# Autodesk Inventor assembly: HAND_asm2
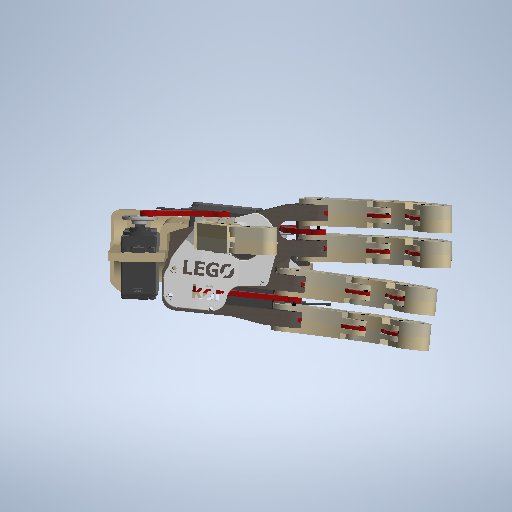
[picture p0: Inventor's stored thumbnail of the model, 512x512]
Saved by Autodesk Inventor 2025.2 (Build 292293000, 293)
## iProperties
Part Number: HAND_asm2
Document SubType Name: Assembly
Designer: esandor
Author: esandor
## Documents named in this file (23)
- C:\Users\esandor\Documents\Inventor\INDACT_EE\again\HAND_THIS_IS_IT.iam
- C:\Users\esandor\Documents\Inventor\INDACT_EE\again\PALM\PALM_base.ipt
- C:\Users\esandor\Documents\Inventor\INDACT_EE\again\HAND\HAND_double_finger_dowel_pin.ipt
- C:\Users\esandor\Documents\Inventor\INDACT_EE\again\FINGER\FIN_phalanx_proximal_top.ipt
- C:\Users\esandor\Documents\Inventor\INDACT_EE\again\FINGER\FIN_dowel_pin_long.ipt
- C:\Users\esandor\Documents\Inventor\INDACT_EE\again\FINGER\FIN_phalanx_proximal_base.ipt
- C:\Users\esandor\Documents\Inventor\INDACT_EE\again\FINGER\FIN_phalanx_media_top.ipt
- C:\Users\esandor\Documents\Inventor\INDACT_EE\again\FINGER\FIN_phalanx_media_base.ipt
- C:\Users\esandor\Documents\Inventor\INDACT_EE\again\FINGER\FIN_dowel_pin_short.ipt
- C:\Users\esandor\Documents\Inventor\INDACT_EE\again\FINGER\FIN_phalanx_distal_top.ipt
- C:\Users\esandor\Documents\Inventor\INDACT_EE\again\FINGER\FIN_phalanx_distal_base.ipt
- C:\Users\esandor\Documents\Inventor\INDACT_EE\again\FINGER\FIN_mech_proximal.ipt
- C:\Users\esandor\Documents\Inventor\INDACT_EE\again\FINGER\FIN_mech_distal.ipt
- C:\Users\esandor\Documents\Inventor\INDACT_EE\again\PALM\PALM_logo.ipt
- C:\Users\esandor\Documents\Inventor\INDACT_EE\again\PALM\PALM_lower_motor_holder.ipt
- C:\Users\esandor\Documents\Inventor\INDACT_EE\again\PALM\PALM_upper_motor_holder.ipt
- C:\Users\esandor\Documents\Inventor\INDACT_EE\again\HAND\HAND_motor_base.ipt
- C:\Users\esandor\Documents\Inventor\INDACT_EE\again\HAND\HAND_motor_top.ipt
- C:\Users\esandor\Documents\Inventor\INDACT_EE\again\HAND\HAND_gyuru.ipt
- C:\Users\esandor\Documents\Inventor\INDACT_EE\again\HAND\HAND_nut.ipt
- C:\Users\esandor\Documents\Inventor\INDACT_EE\again\HAND\HAND_mech_little_finger.ipt
- C:\Users\esandor\Documents\Inventor\INDACT_EE\again\HAND\HAND_mech_thumb_finger.ipt
- C:\Users\esandor\Documents\Inventor\INDACT_EE\again\HAND\HAND_mech_index_finger.ipt
## Components (81 placed, 22 different names)
1. PALM_base:1 — Mate:2, Tangent:2, Insert:2, Insert:9, Insert:11, Mate:24, Tangent:44, Mate:25, Insert:30, Insert:31, Mate:28, Insert:32, Insert:33, Tangent:63, Mate:36, Insert:42, Insert:43, Mate:37, Insert:44, Insert:45
2. FIN_dowel_pin_short:1 — Insert:2, Tangent:5
3. FIN_phalanx_proximal_top:1 — Mate:1, Insert:1, Tangent:1, Mate:2, Tangent:2, Insert:4, Mate:4, Insert:5, Mate:5
4. FIN_phalanx_proximal_base:1 — Mate:1, Insert:1, Tangent:1, Tangent:21
5. FIN_dowel_pin_short:2 — Insert:4, Tangent:9
6. FIN_phalanx_media_top:1 — Mate:3, Tangent:3, Tangent:4, Mate:4, Insert:5, Insert:6, Insert:7, Mate:7
7. FIN_phalanx_media_base:1 — Mate:3, Tangent:3, Tangent:4, Angle:1
8. FIN_dowel_pin_long:2 — Insert:6, Tangent:6
9. FIN_mech_proximal:1 — Tangent:5, Mate:5, Tangent:6
10. FIN_phalanx_distal_top:1 — Mate:6, Tangent:7, Tangent:8, Insert:7, Insert:8
11. FIN_phalanx_distal_base:1 — Mate:6, Tangent:7, Tangent:8, Angle:2
12. FIN_dowel_pin_long:3 — Insert:8, Tangent:10
13. FIN_mech_distal:1 — Mate:7, Tangent:9, Tangent:10
14. FIN_phalanx_proximal_top:2 — Tangent:11, Tangent:12, Mate:8, Insert:9, Insert:12, Insert:13, Mate:10, Insert:17
15. FIN_phalanx_proximal_base:2 — Tangent:11, Tangent:12, Mate:8, Mate:49
16. FIN_dowel_pin_short:3 — Insert:11, Tangent:15
17. FIN_dowel_pin_short:4 — Insert:12, Tangent:19
18. FIN_phalanx_media_top:2 — Insert:13, Insert:14, Insert:15, Mate:12
19. FIN_phalanx_media_base:2 — Angle:1
20. FIN_dowel_pin_long:5 — Insert:14, Tangent:16
21. FIN_mech_proximal:2 — Mate:10, Tangent:15, Tangent:16
22. FIN_phalanx_distal_top:2 — Insert:15, Insert:16
23. FIN_phalanx_distal_base:2 — Angle:2
24. FIN_dowel_pin_long:6 — Insert:16, Tangent:20
25. FIN_mech_distal:3 — Tangent:19, Mate:12, Tangent:20
26. HAND_double_finger_dowel_pin:3 — Insert:17, Tangent:21, Tangent:65
27. FIN_phalanx_proximal_top:3 — Mate:25, Mate:26, Mate:52
28. FIN_phalanx_proximal_base:3 — Tangent:63
29. FIN_dowel_pin_short:6
30. FIN_phalanx_media_top:3
31. FIN_phalanx_media_base:3
32. FIN_dowel_pin_long:7 — Tangent:48
33. FIN_phalanx_distal_top:3
34. FIN_phalanx_distal_base:3
35. FIN_dowel_pin_long:8
36. FIN_mech_distal:4
37. FIN_phalanx_proximal_top:4 — Mate:24, Tangent:44, Mate:27
38. FIN_phalanx_proximal_base:4
39. FIN_dowel_pin_short:8
40. FIN_phalanx_media_top:4
41. FIN_phalanx_media_base:4
42. FIN_dowel_pin_long:9 — Tangent:50
43. FIN_phalanx_distal_top:4
44. FIN_phalanx_distal_base:4
45. FIN_dowel_pin_long:10
46. FIN_mech_distal:5
47. HAND_double_finger_dowel_pin:4 — Tangent:67
48. FIN_dowel_pin_short:9 — Insert:30, Tangent:47
49. FIN_mech_proximal:3 — Mate:26, Tangent:47, Tangent:48
50. FIN_dowel_pin_short:10 — Insert:31, Tangent:49
51. FIN_mech_proximal:4 — Mate:27, Tangent:49, Tangent:50
52. PALM_logo:1 — Mate:28, Insert:32, Insert:33, Mate:35, Insert:40, Insert:41
53. FIN_phalanx_proximal_top:5 — Insert:54
54. FIN_phalanx_proximal_base:5 — Mate:35, Insert:40
55. FIN_dowel_pin_short:12
56. FIN_phalanx_media_top:5
57. FIN_phalanx_media_base:5
58. FIN_dowel_pin_long:11
59. FIN_mech_proximal:5 — Tangent:62
60. FIN_phalanx_distal_top:5
61. FIN_phalanx_distal_base:5
62. FIN_dowel_pin_long:12
63. FIN_mech_distal:6
64. FIN_dowel_pin_short:13 — Insert:41, Tangent:62
65. PALM_lower_motor_holder:1 — Mate:36, Insert:42, Insert:43, Mate:40, Insert:55, Insert:56
66. PALM_upper_motor_holder:1 — Mate:37, Insert:44, Insert:45, Mate:38, Insert:46, Insert:47, Mate:39, Insert:48, Insert:49
67. HAND_motor_base:1 — Mate:38, Insert:46, Insert:47, Rotational:2
68. HAND_motor_base:2 — Mate:39, Insert:48, Insert:49, Rotational:1
69. HAND_motor_base:3 — Mate:40, Insert:55, Insert:56, Rotational:3
70. HAND_motor_top:1 — Rotational:1, Tangent:70
71. HAND_gyuru:1 — Tangent:64, Flush:1, Tangent:65
72. HAND_nut:1 — Mate:50, Mate:51, Tangent:68
73. HAND_mech_little_finger:1 — Mate:50, Mate:51, Tangent:66, Flush:2, Mate:52
74. HAND_mech_thumb_finger:1 — Mate:44, Mate:45, Mate:46, Tangent:71
75. HAND_nut:2 — Mate:44, Tangent:70, Tangent:71
76. HAND_nut:3 — Mate:45, Mate:46, Insert:54
77. HAND_mech_index_finger:1 — Mate:47, Mate:48, Tangent:64, Flush:1, Mate:49
78. HAND_nut:4 — Mate:47, Mate:48, Tangent:69
79. HAND_gyuru:2 — Tangent:66, Flush:2, Tangent:67
80. HAND_motor_top:2 — Rotational:2, Tangent:69
81. HAND_motor_top:3 — Rotational:3, Tangent:68
## Relationships (164: Tangent 60, Insert 50, Mate 47, RevoluteJoint 3, Angle 2, Flush 2)
- Mate:1: FIN_phalanx_proximal_top:1 ↔ FIN_phalanx_proximal_base:1
- Insert:1: FIN_phalanx_proximal_top:1 ↔ FIN_phalanx_proximal_base:1
- Tangent:1: FIN_phalanx_proximal_top:1 ↔ FIN_phalanx_proximal_base:1
- Mate:2: PALM_base:1 ↔ FIN_phalanx_proximal_top:1
- Tangent:2: PALM_base:1 ↔ FIN_phalanx_proximal_top:1
- Insert:2: PALM_base:1 ↔ FIN_dowel_pin_short:1
- Insert:4: FIN_phalanx_proximal_top:1 ↔ FIN_dowel_pin_short:2
- Mate:3: FIN_phalanx_media_top:1 ↔ FIN_phalanx_media_base:1
- Tangent:3: FIN_phalanx_media_top:1 ↔ FIN_phalanx_media_base:1
- Tangent:4: FIN_phalanx_media_top:1 ↔ FIN_phalanx_media_base:1
- Mate:4: FIN_phalanx_proximal_top:1 ↔ FIN_phalanx_media_top:1
- Insert:5: FIN_phalanx_proximal_top:1 ↔ FIN_phalanx_media_top:1
- Insert:6: FIN_phalanx_media_top:1 ↔ FIN_dowel_pin_long:2
- Tangent:5: FIN_dowel_pin_short:1 ↔ FIN_mech_proximal:1
- Mate:5: FIN_phalanx_proximal_top:1 ↔ FIN_mech_proximal:1
- Tangent:6: FIN_dowel_pin_long:2 ↔ FIN_mech_proximal:1
- Mate:6: FIN_phalanx_distal_top:1 ↔ FIN_phalanx_distal_base:1
- Tangent:7: FIN_phalanx_distal_top:1 ↔ FIN_phalanx_distal_base:1
- Tangent:8: FIN_phalanx_distal_top:1 ↔ FIN_phalanx_distal_base:1
- Insert:7: FIN_phalanx_media_top:1 ↔ FIN_phalanx_distal_top:1
- Insert:8: FIN_phalanx_distal_top:1 ↔ FIN_dowel_pin_long:3
- Mate:7: FIN_phalanx_media_top:1 ↔ FIN_mech_distal:1
- Tangent:9: FIN_dowel_pin_short:2 ↔ FIN_mech_distal:1
- Tangent:10: FIN_dowel_pin_long:3 ↔ FIN_mech_distal:1
- Tangent:11: FIN_phalanx_proximal_top:2 ↔ FIN_phalanx_proximal_base:2
- Tangent:12: FIN_phalanx_proximal_top:2 ↔ FIN_phalanx_proximal_base:2
- Mate:8: FIN_phalanx_proximal_top:2 ↔ FIN_phalanx_proximal_base:2
- Insert:9: PALM_base:1 ↔ FIN_phalanx_proximal_top:2
- Insert:11: PALM_base:1 ↔ FIN_dowel_pin_short:3
- Insert:12: FIN_phalanx_proximal_top:2 ↔ FIN_dowel_pin_short:4
- [Mate]: FIN_phalanx_media_top:2 ↔ FIN_phalanx_media_base:2
- [Tangent]: FIN_phalanx_media_top:2 ↔ FIN_phalanx_media_base:2
- [Tangent]: FIN_phalanx_media_top:2 ↔ FIN_phalanx_media_base:2
- Insert:13: FIN_phalanx_proximal_top:2 ↔ FIN_phalanx_media_top:2
- Insert:14: FIN_phalanx_media_top:2 ↔ FIN_dowel_pin_long:5
- Mate:10: FIN_phalanx_proximal_top:2 ↔ FIN_mech_proximal:2
- Tangent:15: FIN_dowel_pin_short:3 ↔ FIN_mech_proximal:2
- Tangent:16: FIN_dowel_pin_long:5 ↔ FIN_mech_proximal:2
- [Mate]: FIN_phalanx_distal_top:2 ↔ FIN_phalanx_distal_base:2
- [Tangent]: FIN_phalanx_distal_top:2 ↔ FIN_phalanx_distal_base:2
- [Tangent]: FIN_phalanx_distal_top:2 ↔ FIN_phalanx_distal_base:2
- Insert:15: FIN_phalanx_media_top:2 ↔ FIN_phalanx_distal_top:2
- Insert:16: FIN_phalanx_distal_top:2 ↔ FIN_dowel_pin_long:6
- Tangent:19: FIN_dowel_pin_short:4 ↔ FIN_mech_distal:3
- Mate:12: FIN_phalanx_media_top:2 ↔ FIN_mech_distal:3
- Tangent:20: FIN_dowel_pin_long:6 ↔ FIN_mech_distal:3
- Insert:17 (-0.43 mm): FIN_phalanx_proximal_top:2 ↔ HAND_double_finger_dowel_pin:3
- Tangent:21: FIN_phalanx_proximal_base:1 ↔ HAND_double_finger_dowel_pin:3
- [Mate]: FIN_phalanx_proximal_top:3 ↔ FIN_phalanx_proximal_base:3
- [Insert]: FIN_phalanx_proximal_top:3 ↔ FIN_phalanx_proximal_base:3
- [Tangent]: FIN_phalanx_proximal_top:3 ↔ FIN_phalanx_proximal_base:3
- [Insert]: FIN_phalanx_proximal_top:3 ↔ FIN_dowel_pin_short:6
- [Mate]: FIN_phalanx_media_top:3 ↔ FIN_phalanx_media_base:3
- [Tangent]: FIN_phalanx_media_top:3 ↔ FIN_phalanx_media_base:3
- [Tangent]: FIN_phalanx_media_top:3 ↔ FIN_phalanx_media_base:3
- [Mate]: FIN_phalanx_proximal_top:3 ↔ FIN_phalanx_media_top:3
- [Insert]: FIN_phalanx_proximal_top:3 ↔ FIN_phalanx_media_top:3
- [Insert]: FIN_phalanx_media_top:3 ↔ FIN_dowel_pin_long:7
- [Mate]: FIN_phalanx_distal_top:3 ↔ FIN_phalanx_distal_base:3
- [Tangent]: FIN_phalanx_distal_top:3 ↔ FIN_phalanx_distal_base:3
- [Tangent]: FIN_phalanx_distal_top:3 ↔ FIN_phalanx_distal_base:3
- [Insert]: FIN_phalanx_media_top:3 ↔ FIN_phalanx_distal_top:3
- [Insert]: FIN_phalanx_distal_top:3 ↔ FIN_dowel_pin_long:8
- [Mate]: FIN_phalanx_media_top:3 ↔ FIN_mech_distal:4
- [Tangent]: FIN_dowel_pin_short:6 ↔ FIN_mech_distal:4
- [Tangent]: FIN_dowel_pin_long:8 ↔ FIN_mech_distal:4
- [Tangent]: FIN_phalanx_proximal_top:4 ↔ FIN_phalanx_proximal_base:4
- [Tangent]: FIN_phalanx_proximal_top:4 ↔ FIN_phalanx_proximal_base:4
- [Mate]: FIN_phalanx_proximal_top:4 ↔ FIN_phalanx_proximal_base:4
- [Insert]: FIN_phalanx_proximal_top:4 ↔ FIN_dowel_pin_short:8
- [Mate]: FIN_phalanx_media_top:4 ↔ FIN_phalanx_media_base:4
- [Tangent]: FIN_phalanx_media_top:4 ↔ FIN_phalanx_media_base:4
- [Tangent]: FIN_phalanx_media_top:4 ↔ FIN_phalanx_media_base:4
- [Insert]: FIN_phalanx_proximal_top:4 ↔ FIN_phalanx_media_top:4
- [Insert]: FIN_phalanx_media_top:4 ↔ FIN_dowel_pin_long:9
- [Mate]: FIN_phalanx_distal_top:4 ↔ FIN_phalanx_distal_base:4
- [Tangent]: FIN_phalanx_distal_top:4 ↔ FIN_phalanx_distal_base:4
- [Tangent]: FIN_phalanx_distal_top:4 ↔ FIN_phalanx_distal_base:4
- [Insert]: FIN_phalanx_media_top:4 ↔ FIN_phalanx_distal_top:4
- [Insert]: FIN_phalanx_distal_top:4 ↔ FIN_dowel_pin_long:10
- [Tangent]: FIN_dowel_pin_short:8 ↔ FIN_mech_distal:5
- [Mate]: FIN_phalanx_media_top:4 ↔ FIN_mech_distal:5
- [Tangent]: FIN_dowel_pin_long:10 ↔ FIN_mech_distal:5
- [Insert] (-0.43 mm): FIN_phalanx_proximal_top:4 ↔ HAND_double_finger_dowel_pin:4
- [Tangent]: FIN_phalanx_proximal_base:3 ↔ HAND_double_finger_dowel_pin:4
- Mate:24: PALM_base:1 ↔ FIN_phalanx_proximal_top:4
- Tangent:44: PALM_base:1 ↔ FIN_phalanx_proximal_top:4
- Mate:25: PALM_base:1 ↔ FIN_phalanx_proximal_top:3
- Insert:30: PALM_base:1 ↔ FIN_dowel_pin_short:9
- Mate:26: FIN_phalanx_proximal_top:3 ↔ FIN_mech_proximal:3
- Tangent:47: FIN_dowel_pin_short:9 ↔ FIN_mech_proximal:3
- Tangent:48: FIN_dowel_pin_long:7 ↔ FIN_mech_proximal:3
- Insert:31: PALM_base:1 ↔ FIN_dowel_pin_short:10
- Mate:27: FIN_phalanx_proximal_top:4 ↔ FIN_mech_proximal:4
- Tangent:49: FIN_dowel_pin_short:10 ↔ FIN_mech_proximal:4
- Tangent:50: FIN_dowel_pin_long:9 ↔ FIN_mech_proximal:4
- Mate:28: PALM_base:1 ↔ PALM_logo:1
- Insert:32: PALM_base:1 ↔ PALM_logo:1
- Insert:33: PALM_base:1 ↔ PALM_logo:1
- [Mate]: FIN_phalanx_proximal_top:5 ↔ FIN_phalanx_proximal_base:5
- [Insert]: FIN_phalanx_proximal_top:5 ↔ FIN_phalanx_proximal_base:5
- [Tangent]: FIN_phalanx_proximal_top:5 ↔ FIN_phalanx_proximal_base:5
- [Insert]: FIN_phalanx_proximal_top:5 ↔ FIN_dowel_pin_short:12
- [Mate]: FIN_phalanx_media_top:5 ↔ FIN_phalanx_media_base:5
- [Tangent]: FIN_phalanx_media_top:5 ↔ FIN_phalanx_media_base:5
- [Tangent]: FIN_phalanx_media_top:5 ↔ FIN_phalanx_media_base:5
- [Mate]: FIN_phalanx_proximal_top:5 ↔ FIN_phalanx_media_top:5
- [Insert]: FIN_phalanx_proximal_top:5 ↔ FIN_phalanx_media_top:5
- [Insert]: FIN_phalanx_media_top:5 ↔ FIN_dowel_pin_long:11
- [Mate]: FIN_phalanx_proximal_top:5 ↔ FIN_mech_proximal:5
- [Tangent]: FIN_dowel_pin_long:11 ↔ FIN_mech_proximal:5
- [Mate]: FIN_phalanx_distal_top:5 ↔ FIN_phalanx_distal_base:5
- [Tangent]: FIN_phalanx_distal_top:5 ↔ FIN_phalanx_distal_base:5
- [Tangent]: FIN_phalanx_distal_top:5 ↔ FIN_phalanx_distal_base:5
- [Insert]: FIN_phalanx_media_top:5 ↔ FIN_phalanx_distal_top:5
- [Insert]: FIN_phalanx_distal_top:5 ↔ FIN_dowel_pin_long:12
- [Mate]: FIN_phalanx_media_top:5 ↔ FIN_mech_distal:6
- [Tangent]: FIN_dowel_pin_short:12 ↔ FIN_mech_distal:6
- [Tangent]: FIN_dowel_pin_long:12 ↔ FIN_mech_distal:6
- Mate:35: PALM_logo:1 ↔ FIN_phalanx_proximal_base:5
- Insert:40: PALM_logo:1 ↔ FIN_phalanx_proximal_base:5
- Insert:41: PALM_logo:1 ↔ FIN_dowel_pin_short:13
- Tangent:62: FIN_mech_proximal:5 ↔ FIN_dowel_pin_short:13
- Tangent:63: PALM_base:1 ↔ FIN_phalanx_proximal_base:3
- Angle:1 (0 deg): FIN_phalanx_media_base:1 ↔ FIN_phalanx_media_base:2
- Angle:2 (0 deg): FIN_phalanx_distal_base:1 ↔ FIN_phalanx_distal_base:2
- Mate:36: PALM_base:1 ↔ PALM_lower_motor_holder:1
- Insert:42: PALM_base:1 ↔ PALM_lower_motor_holder:1
- Insert:43: PALM_base:1 ↔ PALM_lower_motor_holder:1
- Mate:37: PALM_base:1 ↔ PALM_upper_motor_holder:1
- Insert:44: PALM_base:1 ↔ PALM_upper_motor_holder:1
- Insert:45: PALM_base:1 ↔ PALM_upper_motor_holder:1
- Mate:38: PALM_upper_motor_holder:1 ↔ HAND_motor_base:1
- Insert:46: PALM_upper_motor_holder:1 ↔ HAND_motor_base:1
- Insert:47: PALM_upper_motor_holder:1 ↔ HAND_motor_base:1
- Mate:39: PALM_upper_motor_holder:1 ↔ HAND_motor_base:2
- Insert:48: PALM_upper_motor_holder:1 ↔ HAND_motor_base:2
- Insert:49: PALM_upper_motor_holder:1 ↔ HAND_motor_base:2
- Mate:40: PALM_lower_motor_holder:1 ↔ HAND_motor_base:3
- Mate:44: HAND_mech_thumb_finger:1 ↔ HAND_nut:2
- Mate:45: HAND_mech_thumb_finger:1 ↔ HAND_nut:3
- Mate:46: HAND_mech_thumb_finger:1 ↔ HAND_nut:3
- Insert:54: FIN_phalanx_proximal_top:5 ↔ HAND_nut:3
- Mate:47: HAND_mech_index_finger:1 ↔ HAND_nut:4
- Mate:48: HAND_mech_index_finger:1 ↔ HAND_nut:4
- Tangent:64: HAND_gyuru:1 ↔ HAND_mech_index_finger:1
- Flush:1: HAND_gyuru:1 ↔ HAND_mech_index_finger:1
- Tangent:65: HAND_double_finger_dowel_pin:3 ↔ HAND_gyuru:1
- Mate:49: FIN_phalanx_proximal_base:2 ↔ HAND_mech_index_finger:1
- Mate:50: HAND_nut:1 ↔ HAND_mech_little_finger:1
- Mate:51: HAND_nut:1 ↔ HAND_mech_little_finger:1
- Tangent:66: HAND_mech_little_finger:1 ↔ HAND_gyuru:2
- Flush:2: HAND_mech_little_finger:1 ↔ HAND_gyuru:2
- Tangent:67: HAND_double_finger_dowel_pin:4 ↔ HAND_gyuru:2
- Mate:52: FIN_phalanx_proximal_top:3 ↔ HAND_mech_little_finger:1
- Insert:55: PALM_lower_motor_holder:1 ↔ HAND_motor_base:3
- Insert:56: PALM_lower_motor_holder:1 ↔ HAND_motor_base:3
- Tangent:68: HAND_nut:1 ↔ HAND_motor_top:3
- Tangent:69: HAND_nut:4 ↔ HAND_motor_top:2
- Tangent:70: HAND_motor_top:1 ↔ HAND_nut:2
- Tangent:71: HAND_mech_thumb_finger:1 ↔ HAND_nut:2
- Rotational:1 [RevoluteJoint]: HAND_motor_base:2 ↔ HAND_motor_top:1
- Rotational:2 [RevoluteJoint]: HAND_motor_base:1 ↔ HAND_motor_top:2
- Rotational:3 [RevoluteJoint]: HAND_motor_base:3 ↔ HAND_motor_top:3
## Named parameters: d143_d117 = 0 mm, d144_d119 = 0 mm, d145_d120 = 0 mm, d151_d127 = 0 mm, d152_d128 = 0 mm, d153_d129 = 0 mm, d263_d161 = 0 mm, d265_d132 = 0 mm, d266_d133 = 0 mm, d267_d134 = 0 mm, d268_d136 = 0 mm, d269_d137 = 0 mm, d270_d138 = 0 mm, d271_d142 = 0 mm, d272_d143_d117 = 0 mm, d273_d144_d119 = 0 mm, d274_d145_d120 = 0 mm, d275_d146 = 0 mm, d276_d147 = 0 mm, d280_d151_d127 = 0 mm, d281_d152_d128 = 0 mm, d282_d153_d129 = 0 mm, d283_d154 = 0 mm, d284_d155 = 0 mm, d285_d156 = 0 mm, d286_d157 = 0 mm, d287_d158 = 0 mm, d288_d160 = -0.43 mm, d289_d108 = 0 mm, d290_d109 = 0 mm, d291_d110 = 0 mm, d292_d116 = 0 mm, d293_d117 = 0 mm, d294_d119 = 0 mm, d295_d120 = 0 mm, d296_d121 = 0 mm, d297_d122 = 0 mm, d298_d123 = 0 mm, d302_d127 = 0 mm, d303_d128 = 0 mm, d304_d129 = 0 mm, d305_d130 = 0 mm, d306_d131 = 0 mm, d325_d132 = 0 mm, d326_d133 = 0 mm, d327_d134 = 0 mm, d328_d108 = 0 mm, d329_d109 = 0 mm, d330_d110 = 0 mm, d331_d116 = 0 mm, d332_d117 = 0 mm, d333_d119 = 0 mm, d334_d120 = 0 mm, d335_d121 = 0 mm, d336_d122 = 0 mm, d337_d123 = 0 mm, d339_d125 = 0 mm, d340_d126 = 0 mm, d341_d127 = 0 mm, d342_d128 = 0 mm, d343_d129 = 0 mm, d344_d130 = 0 mm, d345_d131 = 0 mm
